# Autodesk Inventor assembly: MK3 Swerve Module FAST
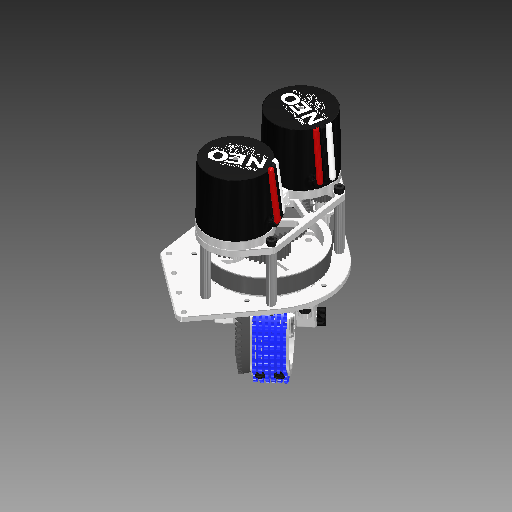
[picture p0: Inventor's stored thumbnail of the model, 512x512]
Saved by Autodesk Inventor 2025 (Build 290162010, 162A)
## iProperties
Created: 2024-07-31
Part Number: MK3 Swerve Module FAST
Document SubType Name: Assembly
Designer: rohan
Author: rohan
## Documents named in this file (9)
- D:\ultimate-hecker\Computer-Aided-Design\FRC-Offseason-Design-Training\Parts Library\Drivetrains\Swerve Modules\MK3\MK3 Swerve Module FAST.iam
- D:\ultimate-hecker\Computer-Aided-Design\FRC-Offseason-Design-Training\Parts Library\Drivetrains\Swerve Modules\MK3\MK3 Turrent Assembly STANDARD.iam
- D:\ultimate-hecker\Computer-Aided-Design\FRC-Offseason-Design-Training\Parts Library\Drivetrains\Swerve Modules\MK3\MK3 Master Structure.iam
- D:\ultimate-hecker\Computer-Aided-Design\FRC-Offseason-Design-Training\Parts Library\Power Transfer\Bearings and Bushings\Bearings\A035XPO_SA035XPO Bearing.ipt
- D:\ultimate-hecker\Computer-Aided-Design\FRC-Offseason-Design-Training\Parts Library\Power Transfer\Belts and Pullies\320-5M-15 Belt.ipt
- D:\ultimate-hecker\Computer-Aided-Design\FRC-Offseason-Design-Training\Parts Library\Power Transfer\Gears (Hex)\32T 32DP Spur Gear 375 Hex (SDS).ipt
- D:\ultimate-hecker\Computer-Aided-Design\FRC-Offseason-Design-Training\Parts Library\Power Transfer\Gears (Motor)\SDS-Steel-Spur-Gear (32DP).ipt
- D:\ultimate-hecker\Computer-Aided-Design\FRC-Offseason-Design-Training\Parts Library\Power Transfer\Gears (Motor)\SDS-Steel-Spur-Gear (20DP, 8mm Bore, 14T, 14T CD).ipt
- D:\ultimate-hecker\Computer-Aided-Design\FRC-Offseason-Design-Training\Parts Library\Hardware\Fasteners\12-24 X .625 Countersunk Screw.ipt
## Components (8 placed, 8 different names)
1. MK3 Turrent Assembly STANDARD:1 [sub-assembly] — Insert:2, Mate:1, Rotation:2, Mate:5
2. MK3 Master Structure:1 [sub-assembly] — Insert:1, Insert:3, Mate:2, Mate:3, Mate:4, Insert:4, Rotation:1, Insert:5
3. A035XPO_SA035XPO Bearing:1 — Insert:1, Insert:2
4. 320-5M-15 Belt:1 — Mate:1, Insert:3
5. 32T 32DP Spur Gear 375 Hex (SDS):1 — Mate:2, Mate:3, Mate:4
6. SDS-Steel-Spur-Gear (32DP):1 — Insert:4, Rotation:1
7. SDS-Steel-Spur-Gear (20DP, 8mm Bore, 14T, 14T CD):1 — Insert:5, Rotation:2
8. 12-24 X .625 Countersunk Screw:1 — Mate:5
## Relationships (12: Insert 5, Mate 5, RelateRotation 2)
- Insert:1: MK3 Master Structure:1 ↔ A035XPO_SA035XPO Bearing:1
- Insert:2: MK3 Turrent Assembly STANDARD:1 ↔ A035XPO_SA035XPO Bearing:1
- Mate:1: MK3 Turrent Assembly STANDARD:1 ↔ 320-5M-15 Belt:1
- Insert:3: MK3 Master Structure:1 ↔ 320-5M-15 Belt:1
- Mate:2: MK3 Master Structure:1 ↔ 32T 32DP Spur Gear 375 Hex (SDS):1
- Mate:3: MK3 Master Structure:1 ↔ 32T 32DP Spur Gear 375 Hex (SDS):1
- Mate:4: MK3 Master Structure:1 ↔ 32T 32DP Spur Gear 375 Hex (SDS):1
- Insert:4: MK3 Master Structure:1 ↔ SDS-Steel-Spur-Gear (32DP):1
- Rotation:1 [RelateRotation] (0.4688 ul): MK3 Master Structure:1 ↔ SDS-Steel-Spur-Gear (32DP):1
- Insert:5: MK3 Master Structure:1 ↔ SDS-Steel-Spur-Gear (20DP, 8mm Bore, 14T, 14T CD):1
- Rotation:2 [RelateRotation] (0.28 ul): MK3 Turrent Assembly STANDARD:1 ↔ SDS-Steel-Spur-Gear (20DP, 8mm Bore, 14T, 14T CD):1
- Mate:5: MK3 Turrent Assembly STANDARD:1 ↔ 12-24 X .625 Countersunk Screw:1
